# Autodesk Inventor assembly: head assy
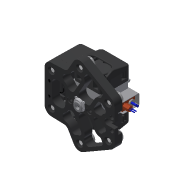
[picture p0: Inventor's stored thumbnail of the model, 180x180]
Saved by Autodesk Inventor 2016 (Build 200138000, 138)
## iProperties
Created: 2016-08-19
Part Number: head assy
Document SubType Name: Assembly
Designer: admin
Author: admin
## Documents named in this file (20)
- C:\Users\Juny\Desktop\Ateam ventures 1805\1806 D3\1612 D3 3D modeling\head assy\head assy.iam
- C:\Users\Juny\Desktop\Ateam ventures 1805\1806 D3\1612 D3 3D modeling\head assy\nozzle_plug.ipt
- C:\Users\Juny\Desktop\Ateam ventures 1805\1806 D3\1612 D3 3D modeling\head assy\tubeclamp male.ipt
- C:\Users\Juny\Desktop\Ateam ventures 1805\1806 D3\1612 D3 3D modeling\head assy\clamp_fixer.ipt
- C:\Users\Juny\Desktop\Ateam ventures 1805\1806 D3\1612 D3 3D modeling\head assy\fan.ipt
- C:\Users\Juny\Desktop\Ateam ventures 1805\1806 D3\1612 D3 3D modeling\head assy\HEAD_cover.ipt
- C:\Users\Juny\Desktop\Ateam ventures 1805\1806 D3\1612 D3 3D modeling\head assy\head_top_plate.ipt
- C:\Users\Juny\Desktop\Ateam ventures 1805\1806 D3\1612 D3 3D modeling\head assy\heat_block.ipt
- C:\Users\Juny\Desktop\Ateam ventures 1805\1806 D3\1612 D3 3D modeling\head assy\heat_cartridge.ipt
- C:\Users\Juny\Desktop\Ateam ventures 1805\1806 D3\1612 D3 3D modeling\head assy\heat_sink.ipt
- C:\Users\Juny\Desktop\Ateam ventures 1805\1806 D3\1612 D3 3D modeling\head assy\m3 6 socket_screw.ipt
- C:\Users\Juny\Desktop\Ateam ventures 1805\1806 D3\1612 D3 3D modeling\head assy\m3 10 socket_screw.ipt
- C:\Users\Juny\Desktop\Ateam ventures 1805\1806 D3\1612 D3 3D modeling\head assy\m3 15 socket_screw.ipt
- C:\Users\Juny\Desktop\Ateam ventures 1805\1806 D3\1612 D3 3D modeling\head assy\magnet.ipt
- C:\Users\Juny\Desktop\Ateam ventures 1805\1806 D3\1612 D3 3D modeling\head assy\fan cover.ipt
- C:\Users\Juny\Desktop\Ateam ventures 1805\1806 D3\1612 D3 3D modeling\head assy\nozzle 0.4.ipt
- C:\Users\Juny\Desktop\Ateam ventures 1805\1806 D3\1612 D3 3D modeling\head assy\nozzle_cover.ipt
- C:\Users\Juny\Desktop\Ateam ventures 1805\1806 D3\1612 D3 3D modeling\head assy\teflon_guide.ipt
- C:\Users\Juny\Desktop\Ateam ventures 1805\1806 D3\1612 D3 3D modeling\head assy\thermistor_ass'y.ipt
- C:\Users\Juny\Desktop\Ateam ventures 1805\1806 D3\1612 D3 3D modeling\head assy\nozzle_cap.ipt
## Components (30 placed, 19 different names)
1. nozzle_plug:1
2. tubeclamp male:1 — Rotational:23
3. clamp_fixer:1 — Rotational:24
4. fan:1 — Rotational:10, Rotational:11, Rotational:16, Rotational:17, Rotational:33
5. HEAD_cover:1 — Rotational:31, Mate:2
6. head_top_plate:1 — Rotational:23, Rotational:24, Rotational:25, Rotational:26, Rotational:30, Rotational:31, Mate:2
7. heat_block:1 — Angle:1, Rotational:22, Mate:4, Mate:5
8. heat_sink:1 — Angle:1, Rotational:10, Rotational:11, Rotational:13, Cylindrical:2, Rotational:36, Angle:2, Angle:3
9. m3 6 socket_screw:1 — Rotational:22
10. m3 10 socket_screw:1 — Rotational:25
11. m3 15 socket_screw:1 — Rotational:14
12. fan:2 — Rotational:13, Rotational:14, Rotational:15, Flush:3, Flush:4
13. m3 15 socket_screw:2 — Rotational:15, Cylindrical:2
14. m3 15 socket_screw:3 — Rotational:16
15. m3 15 socket_screw:4 — Rotational:17
16. m3 10 socket_screw:2 — Rotational:26
17. fan cover:1 — Flush:3, Flush:4
18. fan cover:2 — Rotational:33
19. heat_cartridge:2 — Mate:4
20. nozzle 0.4:1 — Rotational:34, Rotational:35, Mate:6
21. nozzle_cover:1 — Mate:6, Angle:3
22. teflon_guide:1 — Rotational:34
23. thermistor_ass'y:1 — Mate:5
24. nozzle_cap:1 — Rotational:35, Rotational:36, Angle:2
25. magnet:1 — Rotational:30
26. magnet:2
27. magnet:3
28. magnet:4
29. magnet:5
30. magnet:6
## Component patterns: (6 elements, first: magnet:1)
## Relationships (28: RevoluteJoint 18, Mate 4, Angle 3, Flush 2, CylindricalJoint 1)
- Angle:1 (0 deg): heat_block:1 ↔ heat_sink:1
- Rotational:10 [RevoluteJoint]: fan:1 ↔ heat_sink:1
- Rotational:11 [RevoluteJoint]: fan:1 ↔ heat_sink:1
- Rotational:13 [RevoluteJoint]: heat_sink:1 ↔ fan:2
- Rotational:14 [RevoluteJoint]: m3 15 socket_screw:1 ↔ fan:2
- Rotational:15 [RevoluteJoint]: fan:2 ↔ m3 15 socket_screw:2
- Rotational:16 [RevoluteJoint]: fan:1 ↔ m3 15 socket_screw:3
- Rotational:17 [RevoluteJoint]: fan:1 ↔ m3 15 socket_screw:4
- Rotational:22 [RevoluteJoint] (-3 mm): heat_block:1 ↔ m3 6 socket_screw:1
- Rotational:23 [RevoluteJoint] (1 mm): tubeclamp male:1 ↔ head_top_plate:1
- Rotational:24 [RevoluteJoint]: clamp_fixer:1 ↔ head_top_plate:1
- Rotational:25 [RevoluteJoint]: head_top_plate:1 ↔ m3 10 socket_screw:1
- Rotational:26 [RevoluteJoint]: head_top_plate:1 ↔ m3 10 socket_screw:2
- Rotational:30 [RevoluteJoint]: head_top_plate:1 ↔ magnet:1
- Rotational:31 [RevoluteJoint]: HEAD_cover:1 ↔ head_top_plate:1
- Mate:2: HEAD_cover:1 ↔ head_top_plate:1
- Cylindrical:2: heat_sink:1 ↔ m3 15 socket_screw:2
- Flush:3: fan:2 ↔ fan cover:1
- Flush:4: fan:2 ↔ fan cover:1
- Rotational:33 [RevoluteJoint]: fan:1 ↔ fan cover:2
- Mate:4: heat_block:1 ↔ heat_cartridge:2
- Mate:5: heat_block:1 ↔ thermistor_ass'y:1
- Rotational:34 [RevoluteJoint]: nozzle 0.4:1 ↔ teflon_guide:1
- Rotational:35 [RevoluteJoint]: nozzle 0.4:1 ↔ nozzle_cap:1
- Rotational:36 [RevoluteJoint]: heat_sink:1 ↔ nozzle_cap:1
- Angle:2 (0 deg): heat_sink:1 ↔ nozzle_cap:1
- Mate:6: nozzle 0.4:1 ↔ nozzle_cover:1
- Angle:3 (0 deg): heat_sink:1 ↔ nozzle_cover:1
